# Autodesk Inventor assembly: サス
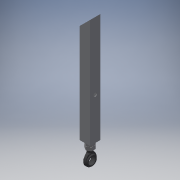
[picture p0: Inventor's stored thumbnail of the model, 180x180]
Saved by Autodesk Inventor 2018 (Build 220112000, 112)
## iProperties
Created: 2017-09-07
Part Number: サス
Material: 一般
Document SubType Name: Assembly
Designer: Kosei
Author: Kosei
## Documents named in this file (5)
- C:\Users\mura5\Documents\RBBR\cart\Rod1.iam
- C:\Users\mura5\Documents\RBBR\cart\Pipe1.ipt
- C:\Users\mura5\Documents\RBBR\cart\hn1_14.ipt
- C:\Users\mura5\Documents\RBBR\cart\iko_POS_14EC\AIS2016\POS 14ECBody.ipt
- C:\Users\mura5\Documents\RBBR\cart\ナット蓋.ipt
## Components (5 placed, 4 different names)
1. Pipe1:1 — 角度:1, リジッド:4
2. hn1_14:2 — リジッド:5, リジッド:6
3. POS 14ECBody:1 — 回転:2, 角度:1
4. hn1_14:3 — 回転:2, リジッド:6
5. ナット蓋:1 — リジッド:4, リジッド:5
## Relationships (6: WeldJoint 4, RevoluteJoint 1, Angle 1)
- [WeldJoint] (15 mm): hn1_14:2 ↔ POS 14ECBody:1
- 回転:2 [RevoluteJoint] (30 mm): POS 14ECBody:1 ↔ hn1_14:3
- 角度:1 [Angle] (0 deg): Pipe1:1 ↔ POS 14ECBody:1
- リジッド:4 [WeldJoint]: Pipe1:1 ↔ ナット蓋:1
- リジッド:5 [WeldJoint]: hn1_14:2 ↔ ナット蓋:1
- リジッド:6 [WeldJoint]: hn1_14:2 ↔ hn1_14:3
